# Autodesk Inventor assembly: motor
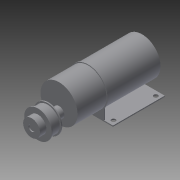
[picture p0: Inventor's stored thumbnail of the model, 180x180]
Saved by Autodesk Inventor 2015 (Build 190159000, 159)
## iProperties
Created: 2015-08-03
Part Number: motor
Document SubType Name: Assembly
Designer: astralien3000
Author: astralien3000
## Documents named in this file (3)
- C:\Users\astralien3000\Desktop\ceres\meca\v2016\motor.iam
- C:\Users\astralien3000\Desktop\ceres\meca\lib\motor\mfa_970d471.ipt
- C:\Users\astralien3000\Desktop\ceres\meca\lib\struct\poulie_conrad_209515.ipt
## Components (2 placed, 2 different names)
1. mfa_970d471:1 — Placage:1, Placage:2
2. poulie_conrad_209515:1 — Placage:1, Placage:2
## Relationships (2: Mate 2)
- Placage:1 [Mate]: mfa_970d471:1 ↔ poulie_conrad_209515:1
- Placage:2 [Mate]: mfa_970d471:1 ↔ poulie_conrad_209515:1
